# Autodesk Inventor assembly: TR2 Arm
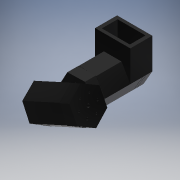
[picture p0: Inventor's stored thumbnail of the model, 180x180]
Saved by Autodesk Inventor 2017 (Build 210142000, 142)
## iProperties
Created: 2018-10-11
Part Number: TR2 Arm
Document SubType Name: Assembly
Designer: Zach
Author: Zach
## Documents named in this file (3)
- C:\Users\Administrator\Documents\GitHub\tr2\Arm\Arm.iam
- C:\Users\Administrator\Documents\GitHub\tr2\Arm\TARM01.ipt
- C:\Users\Administrator\Documents\GitHub\tr2\Arm Actuator\Arm Actuator.iam
## Components (3 placed, 2 different names)
1. TARM01:1 — Mate:9, Mate:10, Mate:11
2. Arm Actuator:1 [sub-assembly] — Mate:9, Mate:10, Mate:11, Mate:12
3. Arm Actuator:2 [sub-assembly] — Mate:12
## Relationships (4: Mate 4)
- Mate:9: TARM01:1 ↔ Arm Actuator:1
- Mate:10: TARM01:1 ↔ Arm Actuator:1
- Mate:11: TARM01:1 ↔ Arm Actuator:1
- Mate:12: Arm Actuator:1 ↔ Arm Actuator:2
